# Autodesk Inventor assembly: pince
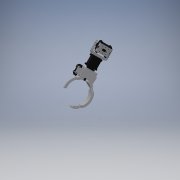
[picture p0: Inventor's stored thumbnail of the model, 180x180]
Saved by Autodesk Inventor 2017 (Build 210142000, 142)
## iProperties
Created: 2017-04-16
Part Number: pince
Document SubType Name: Assembly
Designer: franc
Author: franc
## Documents named in this file (9)
- C:\Users\franc\Desktop\EsialRobotik\Mecanique\robot-2017\pince\pince.iam
- C:\Users\franc\Desktop\EsialRobotik\Mecanique\robot-2017\pince\fixationPince.iam
- C:\Users\franc\Desktop\EsialRobotik\Mecanique\robot-2017\pince\pinceDroite.iam
- C:\Users\franc\Desktop\EsialRobotik\Mecanique\robot-2017\pince\pinceGaucheMini.iam
- C:\Users\franc\Desktop\EsialRobotik\Mecanique\robot-2017\AX12-minerai\ax12_wheel.ipt
- C:\Users\franc\Desktop\EsialRobotik\Mecanique\robot-2017\AX12-minerai\ax12_box.ipt
- C:\Users\franc\Desktop\EsialRobotik\Mecanique\robot-2017\AX12-minerai\ax12_cog.ipt
- C:\Users\franc\Desktop\EsialRobotik\Mecanique\robot-2017\AX12-minerai\F2.ipt
- C:\Users\franc\Desktop\EsialRobotik\Mecanique\robot-2017\AX12-minerai\F3.ipt
## Components (14 placed, 8 different names)
1. fixationPince:1 [sub-assembly] — Mate:1, Mate:2, Mate:3, Mate:4, Mate:8, Mate:9, Mate:10, Mate:11
2. pinceDroite:1 [sub-assembly] — Mate:3, Mate:4, Mate:5, Mate:6, Mate:7
3. pinceGaucheMini:1 [sub-assembly] — Mate:1, Mate:2
4. ax12_wheel:1 — Mate:5, Mate:6, Mate:7
5. ax12_box:1 — Mate:8
6. ax12_cog:1
7. ax12_wheel:2 — Mate:9, Mate:10, Mate:11
8. ax12_box:2 — Mate:20, Mate:21, Mate:22
9. ax12_cog:2
10. ax12_wheel:3
11. ax12_box:3 — Mate:17, Mate:18, Mate:19
12. ax12_cog:3
13. F2:1 — Mate:20, Mate:21, Mate:22
14. F3:1 — Mate:17, Mate:18, Mate:19
## Relationships (23: Mate 20, Insert 3)
- Mate:1: fixationPince:1 ↔ pinceGaucheMini:1
- Mate:2: fixationPince:1 ↔ pinceGaucheMini:1
- Mate:3: fixationPince:1 ↔ pinceDroite:1
- Mate:4: fixationPince:1 ↔ pinceDroite:1
- [Insert]: ax12_wheel:1 ↔ ax12_box:1
- Mate:5: pinceDroite:1 ↔ ax12_wheel:1
- Mate:6: pinceDroite:1 ↔ ax12_wheel:1
- Mate:7: pinceDroite:1 ↔ ax12_wheel:1
- Mate:8: fixationPince:1 ↔ ax12_box:1
- [Insert]: ax12_wheel:2 ↔ ax12_box:2
- Mate:9: fixationPince:1 ↔ ax12_wheel:2
- Mate:10: fixationPince:1 ↔ ax12_wheel:2
- Mate:11: fixationPince:1 ↔ ax12_wheel:2
- [Insert]: ax12_wheel:3 ↔ ax12_box:3
- [Mate]: ax12_wheel:3 ↔ F2:1
- [Mate]: ax12_wheel:3 ↔ F2:1
- [Mate]: ax12_wheel:3 ↔ F2:1
- Mate:17: ax12_box:3 ↔ F3:1
- Mate:18: ax12_box:3 ↔ F3:1
- Mate:19: ax12_box:3 ↔ F3:1
- Mate:20: ax12_box:2 ↔ F2:1
- Mate:21: ax12_box:2 ↔ F2:1
- Mate:22: ax12_box:2 ↔ F2:1
## Named parameters: d4_d1 = 0 mm, d9_d1 = 0 mm, d16_d1 = 0 mm
